# Autodesk Inventor assembly: M5 Screw with Tee Nut_MIR
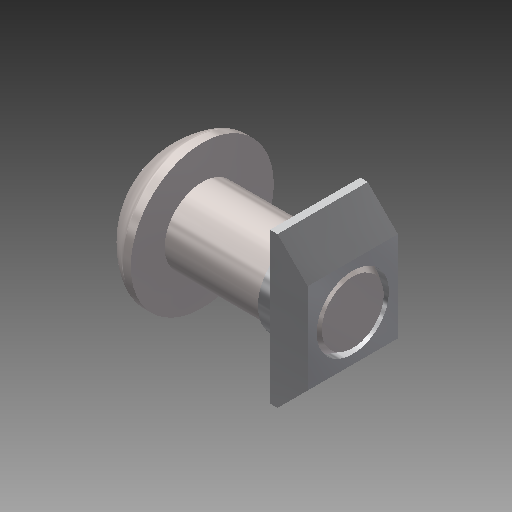
[picture p0: Inventor's stored thumbnail of the model, 512x512]
Saved by Autodesk Inventor 2017 (Build 210142000, 142)
## iProperties
Created: 2014-02-18
Part Number: M5 Screw with Tee Nut_MIR
Document SubType Name: Assembly
Designer: umr
Author: umr
Sending System: SolidWorks 2014
Last Author: Rory
Last Saved: 2016-05-20
## Documents named in this file (3)
- D:\SeniorProject\Models2\Elevator\M5 Screw with Tee Nut_MIR.iam
- D:\SeniorProject\Models2\Elevator\Tee Nut_MIR.ipt
- D:\SeniorProject\Models2\Elevator\M5 Screw_MIR.ipt
## Components (2 placed, 2 different names)
1. Tee Nut_MIR:1 — Flush:1, Mate:2
2. M5 Screw_MIR:1 — Flush:1, Mate:2
## Relationships (2: Flush 1, Mate 1)
- Flush:1: Tee Nut_MIR:1 ↔ M5 Screw_MIR:1
- Mate:2: Tee Nut_MIR:1 ↔ M5 Screw_MIR:1
